# Autodesk Inventor assembly: Assembly
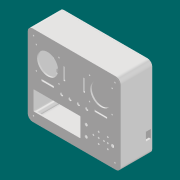
[picture p0: Inventor's stored thumbnail of the model, 180x180]
Saved by Autodesk Inventor 2020.1 (Build 241239000, 239)
## iProperties
Created: 2019-07-23
Part Number: Assembly
Document SubType Name: Assembly
Designer: Pluscrafter
Author: Pluscrafter
## Documents named in this file (4)
- D:\Pluscrafter\Documents\SHARKSKY\02_RCTransmitter\CAD\Assembly.iam
- D:\Pluscrafter\Documents\SHARKSKY\02_RCTransmitter\CAD\Back.ipt
- D:\Pluscrafter\Documents\SHARKSKY\02_RCTransmitter\CAD\Housing.ipt
- D:\Pluscrafter\Documents\SHARKSKY\02_RCTransmitter\CAD\Front.ipt
## Components (3 placed, 3 different names)
1. Back:1 — Mate:1, Mate:2
2. Front:1 — Mate:3, Mate:4
3. Housing:1 — Mate:1, Mate:2, Mate:3, Mate:4
## Relationships (4: Mate 4)
- Mate:1: Back:1 ↔ Housing:1
- Mate:2: Back:1 ↔ Housing:1
- Mate:3: Front:1 ↔ Housing:1
- Mate:4: Front:1 ↔ Housing:1
